# Autodesk Inventor assembly: HbButtonU01
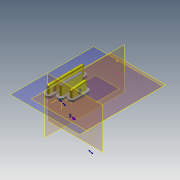
[picture p0: Inventor's stored thumbnail of the model, 180x180]
Saved by Autodesk Inventor 2015 SP1 (Build 190203100, 203)
## iProperties
Created: 2016-01-24
Part Number: HbButtonU01
Document SubType Name: Assembly
Designer: Yamaura
Author: Yamaura
## Documents named in this file (6)
- C:\Users\Yamaura\Documents\GitHub\HACKberry\HACKberry-hardware\3D\Inventor\Parts\HbButtonU01.iam
- C:\Users\Yamaura\Documents\GitHub\HACKberry\HACKberry-hardware\3D\Inventor\Parts\HbFingerLockButton05.ipt
- C:\Users\Yamaura\Documents\GitHub\HACKberry\HACKberry-hardware\3D\Inventor\Parts\HbMaxButton05.ipt
- C:\Users\Yamaura\Documents\GitHub\HACKberry\HACKberry-hardware\3D\Inventor\Parts\HbMinButton05.ipt
- C:\Users\Yamaura\Documents\GitHub\HACKberry\HACKberry-hardware\3D\Inventor\Parts\HbThumbButton05.ipt
- C:\Users\Yamaura\Documents\GitHub\HACKberry\HACKberry-hardware\3D\Inventor\Parts\HbPowerLever05.ipt
## Components (5 placed, 5 different names)
1. HbFingerLockButton05:1 — メイト:12, メイト:13
2. HbMaxButton05:1 — メイト:4, メイト:7, メイト:8
3. HbMinButton05:1 — メイト:3, メイト:8, メイト:9, メイト:10
4. HbThumbButton05:1 — メイト:2, メイト:9, メイト:11
5. HbPowerLever05:1 — メイト:1, メイト:6, メイト:7, メイト:10, メイト:11, メイト:12
## Relationships (12: Mate 12)
- メイト:1 [Mate]: HbPowerLever05:1
- メイト:2 [Mate]: HbThumbButton05:1
- メイト:3 [Mate]: HbMinButton05:1
- メイト:4 [Mate]: HbMaxButton05:1
- メイト:6 [Mate]: HbPowerLever05:1
- メイト:7 [Mate] (0.3 mm): HbMaxButton05:1 ↔ HbPowerLever05:1
- メイト:8 [Mate] (0.3 mm): HbMaxButton05:1 ↔ HbMinButton05:1
- メイト:9 [Mate] (0.3 mm): HbMinButton05:1 ↔ HbThumbButton05:1
- メイト:10 [Mate] (0.3 mm): HbMinButton05:1 ↔ HbPowerLever05:1
- メイト:11 [Mate] (0.3 mm): HbThumbButton05:1 ↔ HbPowerLever05:1
- メイト:12 [Mate] (0.3 mm): HbFingerLockButton05:1 ↔ HbPowerLever05:1
- メイト:13 [Mate]: HbFingerLockButton05:1
